# Autodesk Inventor assembly: ensamble
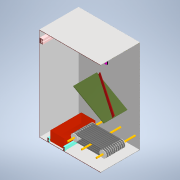
[picture p0: Inventor's stored thumbnail of the model, 180x180]
Saved by Autodesk Inventor 2021.1 (Build 251245000, 245)
## iProperties
Created: 2020-12-31
Part Number: ensamble
Document SubType Name: Assembly
Designer: Bolisteward
Author: Bolisteward
## Documents named in this file (8)
- D:\Inventor works\Embebidos\ensamble.iam
- D:\Inventor works\Embebidos\caja.ipt
- D:\Inventor works\Embebidos\rueda de enganche.ipt
- D:\Inventor works\Embebidos\gancho.ipt
- D:\Inventor works\Embebidos\caja de mascarilllas.ipt
- D:\Inventor works\Embebidos\compuerta.ipt
- D:\Inventor works\Embebidos\palanca.ipt
- D:\Inventor works\Embebidos\ensamble\Design Accelerator\V-Belt transmission1.iam
## Components (7 placed, 7 different names)
1. caja:1 — Mate:1, Flush:1, Mate:2, Mate:3, Mate:4, Mate:5, Mate:6, Mate:7, Mate:8, Mate:9
2. rueda de enganche:1 — Mate:1, Flush:1
3. gancho:1 — Mate:2, Mate:3
4. caja de mascarilllas:1 — Mate:4, Mate:5
5. compuerta:1 — Mate:6, Mate:7
6. palanca:1 — Mate:8, Mate:9
7. V-Belt transmission:1 [sub-assembly]
## Relationships (10: Mate 9, Flush 1)
- Mate:1: caja:1 ↔ rueda de enganche:1
- Flush:1: caja:1 ↔ rueda de enganche:1
- Mate:2: caja:1 ↔ gancho:1
- Mate:3: caja:1 ↔ gancho:1
- Mate:4: caja:1 ↔ caja de mascarilllas:1
- Mate:5: caja:1 ↔ caja de mascarilllas:1
- Mate:6: caja:1 ↔ compuerta:1
- Mate:7 (40 mm): caja:1 ↔ compuerta:1
- Mate:8: caja:1 ↔ palanca:1
- Mate:9: caja:1 ↔ palanca:1
